# Autodesk Inventor assembly: Assembly1
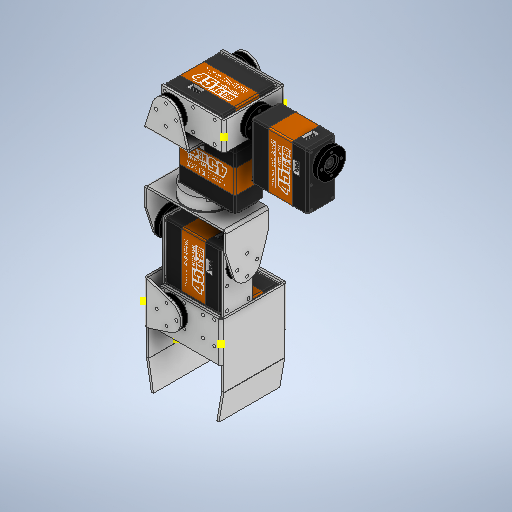
[picture p0: Inventor's stored thumbnail of the model, 512x512]
Saved by Autodesk Inventor 2025.2 (Build 292293000, 293)
## iProperties
Created: 2025-05-12
Part Number: Assembly1
Document SubType Name: Assembly
Designer: LG
Author: LG
## Documents named in this file (14)
- C:\Users\LG\Desktop\RHp_Humanoid_ver1\Assembly\6_right_Arm.iam
- C:\Users\LG\Desktop\RHp_Humanoid_ver1\Part\Frame\Arm\axis_19_top_frame.ipt
- C:\Users\LG\Desktop\RHp_Humanoid_ver1\Part\HTD-45H, Horn\HTD-45H\HTD-45H.ipt
- C:\Users\LG\Desktop\RHp_Humanoid_ver1\Part\HTD-45H, Horn\Horn\Top Horn.ipt
- C:\Users\LG\Desktop\RHp_Humanoid_ver1\Part\Frame\Arm\axis_21_top_frame.ipt
- C:\Users\LG\Desktop\RHp_Humanoid_ver1\Part\Frame\Arm\axis_21_bottom_frame.ipt
- C:\Users\LG\Desktop\RHp_Humanoid_ver1\Part\Frame\Arm\axis_23_bottom_frame.ipt
- C:\Users\LG\Desktop\RHp_Humanoid_ver1\Part\HTD-45H, Horn\Horn\Bottom Horn.ipt
- C:\Users\LG\Desktop\RHp_Humanoid_ver1\Part\Frame\Arm\axis_20_bottom_frame.ipt
- C:\Users\LG\Desktop\RHp_Humanoid_ver1\Part\Bolt, Bearing, Nut, Washer\2030 Teflon Sheet.ipt
- C:\Users\LG\Desktop\RHp_Humanoid_ver1\Part\HTD-45H, Horn\HTD-45H\HTD-45H.iam
- C:\Users\LG\Desktop\RHp_Humanoid_ver1\Part\Frame\Arm\axis_23_top_frame.ipt
- C:\Users\LG\Desktop\RHp_Humanoid_ver1\Part\Frame\Arm\axis_22_top_frame.ipt
- C:\Users\LG\Desktop\RHp_Humanoid_ver1\Part\Frame\Arm\axis_22_bottom_frame.ipt
## Components (24 placed, 12 different names)
1. Bottom Horn:2 — Mate:54, Mate:55, Flush:31
2. HTD-45H:3 [sub-assembly] — Mate:54, Mate:55, Flush:31, Mate:59, Mate:60, Mate:62, Rotational:1
3. Top Horn:6 — Rotational:1, Mate:86, Flush:43, Flush:44
4. axis_19_top_frame:1 — Mate:86, Flush:43, Flush:44, Mate:109, Flush:62, Mate:110
5. Bottom Horn:1 — Flush:28, Mate:41, Mate:42
6. HTD-45H:1 — Flush:28, Mate:41, Mate:42, Rotational:2, Mate:109, Flush:62, Mate:110
7. Top Horn:7 — Rotational:2, Mate:87, Mate:88, Flush:45
8. axis_20_bottom_frame:1 — Mate:87, Mate:88, Flush:45, Mate:89, Mate:90, Flush:46
9. HTD-45H:2 — Mate:13, Mate:89, Mate:90, Flush:46, Rotational:3, Mate:107, Flush:60
10. Top Horn:8 — Rotational:3, Mate:92, Flush:49, Mate:93, Mate:112, Mate:113
11. axis_21_top_frame:1 — Mate:13, Mate:91, Mate:107, Flush:60
12. 2030 Teflon Sheet:1 — Mate:91, Mate:92, Flush:49, Mate:122, Mate:123, Mate:124
13. 2030 Teflon Sheet:2 — Mate:122, Mate:123, Mate:124
14. axis_21_bottom_frame:1 — Mate:93, Mate:97, Mate:111, Flush:63, Mate:112, Mate:113
15. Bottom Horn:3 — Mate:65, Mate:66, Flush:32
16. HTD-45H:4 [sub-assembly] — Mate:65, Mate:66, Flush:32, Rotational:4, Mate:99, Flush:64, Mate:115, Mate:117, Flush:67
17. Top Horn:9 — Rotational:4, Mate:97, Mate:111, Flush:63
18. axis_22_top_frame:1 — Mate:115, Mate:116, Mate:117, Mate:118, Mate:121
19. axis_22_bottom_frame:1 — Mate:118, Mate:119, Flush:65, Mate:120, Flush:68
20. Bottom Horn:4 — Mate:75, Mate:76, Flush:34
21. HTD-45H:5 [sub-assembly] — Mate:75, Mate:76, Flush:34, Mate:99, Rotational:5, Flush:64, Mate:116, Mate:119, Flush:65, Flush:67
22. Top Horn:10 — Rotational:5, Flush:58, Flush:59, Mate:106
23. axis_23_bottom_frame:1 — Flush:58, Flush:59, Mate:106
24. axis_23_top_frame:1 — Mate:120, Mate:121, Flush:68
## Relationships (62: Mate 39, Flush 18, RevoluteJoint 5)
- Mate:13: HTD-45H:2 ↔ axis_21_top_frame:1
- Flush:28: Bottom Horn:1 ↔ HTD-45H:1
- Mate:41: Bottom Horn:1 ↔ HTD-45H:1
- Mate:42: Bottom Horn:1 ↔ HTD-45H:1
- Mate:54: Bottom Horn:2 ↔ HTD-45H:3
- Mate:55: Bottom Horn:2 ↔ HTD-45H:3
- Flush:31: Bottom Horn:2 ↔ HTD-45H:3
- Mate:59: HTD-45H:3
- Mate:60: HTD-45H:3
- Mate:62: HTD-45H:3
- Mate:65: Bottom Horn:3 ↔ HTD-45H:4
- Mate:66: Bottom Horn:3 ↔ HTD-45H:4
- Flush:32: Bottom Horn:3 ↔ HTD-45H:4
- Mate:75: Bottom Horn:4 ↔ HTD-45H:5
- Mate:76: Bottom Horn:4 ↔ HTD-45H:5
- Flush:34: Bottom Horn:4 ↔ HTD-45H:5
- Rotational:1 [RevoluteJoint]: HTD-45H:3 ↔ Top Horn:6
- Mate:86: Top Horn:6 ↔ axis_19_top_frame:1
- Flush:43: Top Horn:6 ↔ axis_19_top_frame:1
- Flush:44: Top Horn:6 ↔ axis_19_top_frame:1
- Rotational:2 [RevoluteJoint]: HTD-45H:1 ↔ Top Horn:7
- Mate:87: Top Horn:7 ↔ axis_20_bottom_frame:1
- Mate:88: Top Horn:7 ↔ axis_20_bottom_frame:1
- Flush:45 (-14.5 mm): Top Horn:7 ↔ axis_20_bottom_frame:1
- Mate:89: axis_20_bottom_frame:1 ↔ HTD-45H:2
- Mate:90: axis_20_bottom_frame:1 ↔ HTD-45H:2
- Flush:46: axis_20_bottom_frame:1 ↔ HTD-45H:2
- Rotational:3 [RevoluteJoint]: HTD-45H:2 ↔ Top Horn:8
- Mate:91: axis_21_top_frame:1 ↔ 2030 Teflon Sheet:1
- Mate:92: Top Horn:8 ↔ 2030 Teflon Sheet:1
- Flush:49: Top Horn:8 ↔ 2030 Teflon Sheet:1
- Mate:93: Top Horn:8 ↔ axis_21_bottom_frame:1
- Rotational:4 [RevoluteJoint]: HTD-45H:4 ↔ Top Horn:9
- Mate:97 (26.43 mm): axis_21_bottom_frame:1 ↔ Top Horn:9
- Mate:99: HTD-45H:4 ↔ HTD-45H:5
- Rotational:5 [RevoluteJoint]: HTD-45H:5 ↔ Top Horn:10
- Flush:58 (-14.43 mm): Top Horn:10 ↔ axis_23_bottom_frame:1
- Flush:59: Top Horn:10 ↔ axis_23_bottom_frame:1
- Mate:106: Top Horn:10 ↔ axis_23_bottom_frame:1
- Mate:107: HTD-45H:2 ↔ axis_21_top_frame:1
- Flush:60: HTD-45H:2 ↔ axis_21_top_frame:1
- Mate:109 (2.5 mm): axis_19_top_frame:1 ↔ HTD-45H:1
- Flush:62: axis_19_top_frame:1 ↔ HTD-45H:1
- Mate:110: axis_19_top_frame:1 ↔ HTD-45H:1
- Mate:111: axis_21_bottom_frame:1 ↔ Top Horn:9
- Flush:63: axis_21_bottom_frame:1 ↔ Top Horn:9
- Mate:112: Top Horn:8 ↔ axis_21_bottom_frame:1
- Mate:113: Top Horn:8 ↔ axis_21_bottom_frame:1
- Flush:64: HTD-45H:4 ↔ HTD-45H:5
- Mate:115: HTD-45H:4 ↔ axis_22_top_frame:1
- Mate:116 (5 mm): axis_22_top_frame:1 ↔ HTD-45H:5
- Mate:117: HTD-45H:4 ↔ axis_22_top_frame:1
- Mate:118: axis_22_top_frame:1 ↔ axis_22_bottom_frame:1
- Mate:119: axis_22_bottom_frame:1 ↔ HTD-45H:5
- Flush:65: axis_22_bottom_frame:1 ↔ HTD-45H:5
- Mate:120: axis_22_bottom_frame:1 ↔ axis_23_top_frame:1
- Mate:121: axis_22_top_frame:1 ↔ axis_23_top_frame:1
- Mate:122: 2030 Teflon Sheet:1 ↔ 2030 Teflon Sheet:2
- Mate:123: 2030 Teflon Sheet:1 ↔ 2030 Teflon Sheet:2
- Mate:124: 2030 Teflon Sheet:1 ↔ 2030 Teflon Sheet:2
- Flush:67: HTD-45H:4 ↔ HTD-45H:5
- Flush:68: axis_22_bottom_frame:1 ↔ axis_23_top_frame:1
